# Autodesk Inventor assembly: hph_002
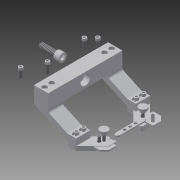
[picture p0: Inventor's stored thumbnail of the model, 180x180]
Saved by Autodesk Inventor 2014 (Build 180170000, 170)
## iProperties
Created: 2014-03-27
Part Number: hph_002
Document SubType Name: Assembly
Designer: stephenholtz
Author: stephenholtz
## Documents named in this file (11)
- C:\Users\stephenholtz\Dropbox\grad_school_docs\sabatini_lab_rotation\headpost_design\hph_001_full.iam
- C:\Users\stephenholtz\Dropbox\grad_school_docs\sabatini_lab_rotation\headpost_design\hph_C_001.ipt
- C:\Users\stephenholtz\Dropbox\grad_school_docs\sabatini_lab_rotation\headpost_design\hph_B_001.ipt
- C:\Users\stephenholtz\Dropbox\grad_school_docs\sabatini_lab_rotation\headpost_design\hph_A_001_left.ipt
- C:\Users\stephenholtz\Dropbox\grad_school_docs\sabatini_lab_rotation\headpost_design\hph_A_001_right.ipt
- C:\Users\stephenholtz\Dropbox\grad_school_docs\sabatini_lab_rotation\headpost_design\hph_D_001.ipt
- C:\Users\stephenholtz\Dropbox\grad_school_docs\sabatini_lab_rotation\headpost_design\hp_thick_001.ipt
- C:\Users\stephenholtz\Dropbox\grad_school_docs\sabatini_lab_rotation\headpost_design\standard_parts\4_-_40_hex_cap_screw.ipt
- C:\Users\stephenholtz\Dropbox\grad_school_docs\sabatini_lab_rotation\headpost_design\standard_parts\4_-_40_set_screw.ipt
- C:\Users\stephenholtz\Dropbox\grad_school_docs\sabatini_lab_rotation\headpost_design\standard_parts\wide_dia_knurled_shoulder_screw.ipt
- C:\Users\stephenholtz\Dropbox\grad_school_docs\sabatini_lab_rotation\headpost_design\standard_parts\1_4_-_20_hex_cap_screw.ipt
## Components (21 placed, 10 different names)
1. hph_C_001:1 — Mate:1, Mate:2, Mate:3, Mate:4, Flush:1, Flush:2
2. hph_B_001:1 — Mate:1, Mate:3, Flush:1, Insert:1, Flush:3
3. hph_B_001:2 — Mate:2, Mate:4, Flush:2, Insert:2, Flush:4
4. hph_A_001_left:1 — Insert:2, Flush:4
5. hph_A_001_right:1 — Insert:1, Flush:3
6. hph_D_001:1
7. hph_D_001:2
8. hp_thick_001:1
9. 4_-_40_hex_cap_screw:1
10. 4_-_40_hex_cap_screw:2
11. 4_-_40_hex_cap_screw:3
12. 4_-_40_hex_cap_screw:4
13. 4_-_40_hex_cap_screw:5
14. 4_-_40_hex_cap_screw:6
15. 4_-_40_hex_cap_screw:7
16. 4_-_40_hex_cap_screw:8
17. 4_-_40_set_screw:1
18. 4_-_40_set_screw:2
19. wide_dia_knurled_shoulder_screw:1
20. wide_dia_knurled_shoulder_screw:2
21. 1_4_-_20_hex_cap_screw:1
## Relationships (10: Mate 4, Flush 4, Insert 2)
- Mate:1: hph_C_001:1 ↔ hph_B_001:1
- Mate:2: hph_C_001:1 ↔ hph_B_001:2
- Mate:3: hph_C_001:1 ↔ hph_B_001:1
- Mate:4: hph_C_001:1 ↔ hph_B_001:2
- Flush:1: hph_C_001:1 ↔ hph_B_001:1
- Flush:2: hph_C_001:1 ↔ hph_B_001:2
- Insert:1: hph_B_001:1 ↔ hph_A_001_right:1
- Flush:3: hph_B_001:1 ↔ hph_A_001_right:1
- Insert:2: hph_B_001:2 ↔ hph_A_001_left:1
- Flush:4: hph_B_001:2 ↔ hph_A_001_left:1
